# Autodesk Inventor assembly: 90deg Corner (OpenBuilds)
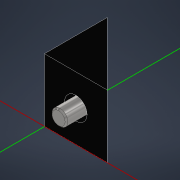
[picture p0: Inventor's stored thumbnail of the model, 180x180]
Saved by Autodesk Inventor 2022 (Build 260153000, 153)
## iProperties
Created: 2022-03-06
Part Number: 90deg Corner (OpenBuilds)
Document SubType Name: Assembly
Designer: sleib
Author: sleib
## Documents named in this file (4)
- C:\Users\sleib\Projekte\Voron-2\CAD\Inventor\90deg Corner (OpenBuilds).iam
- C:\Users\sleib\Projekte\Voron-2\CAD\Inventor\M5 Spacer (1mm).ipt
- C:\Users\sleib\Projekte\Voron-2\CAD\Inventor\M5x10 BHCS.ipt
- C:\Users\sleib\Projekte\Voron-2\CAD\Inventor\Frame Corner (90deg).ipt
## Components (5 placed, 4 different names)
1. Frame Corner (90deg) — Passend:1, Passend:2, Passend:3, Passend:4
2. M5 1mm Spacer:9 — Passend:1, Passend:2, Passend:5, Passend:6
3. M5 Spacer (1mm):2 — Passend:3, Passend:4, Passend:7, Passend:8
4. M5x10 BHCS:2 — Passend:5, Passend:6
5. M5x10 BHCS:70 — Passend:7, Passend:8
## Relationships (8: Mate 8)
- Passend:1 [Mate]: Frame Corner (90deg) ↔ M5 1mm Spacer:9
- Passend:2 [Mate]: Frame Corner (90deg) ↔ M5 1mm Spacer:9
- Passend:3 [Mate]: Frame Corner (90deg) ↔ M5 Spacer (1mm):2
- Passend:4 [Mate]: Frame Corner (90deg) ↔ M5 Spacer (1mm):2
- Passend:5 [Mate]: M5 1mm Spacer:9 ↔ M5x10 BHCS:2
- Passend:6 [Mate]: M5 1mm Spacer:9 ↔ M5x10 BHCS:2
- Passend:7 [Mate]: M5 Spacer (1mm):2 ↔ M5x10 BHCS:70
- Passend:8 [Mate]: M5 Spacer (1mm):2 ↔ M5x10 BHCS:70
